# Autodesk Inventor assembly: HubAndAxel
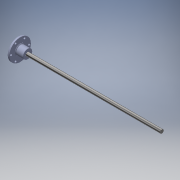
[picture p0: Inventor's stored thumbnail of the model, 180x180]
Saved by Autodesk Inventor 2017 (Build 210142000, 142)
## iProperties
Created: 2016-02-07
Part Number: HubAndAxel
Document SubType Name: Assembly
Designer: steele
Author: steele
## Documents named in this file (3)
- C:\snobotics\CAD-Development\robSteele\SnoBotics2016\2016-05-05-ShooterPrototype\HubAndAxel.iam
- C:\snobotics\CAD-Development\robSteele\SnoBotics2016\AM Parts\am-0134a+375+Key+Hub+r2.ipt
- C:\snobotics\CAD-Development\robSteele\SnoBotics2016\2016-05-05-ShooterPrototype\SteelRodForShooter.ipt
## Components (2 placed, 2 different names)
1. SteelRodForShooter:1 — Insert:5
2. am-0134a+375+Key+Hub+r2:1 — Insert:5
## Relationships (1: Insert 1)
- Insert:5: SteelRodForShooter:1 ↔ am-0134a+375+Key+Hub+r2:1
